# Autodesk Inventor assembly: AK80
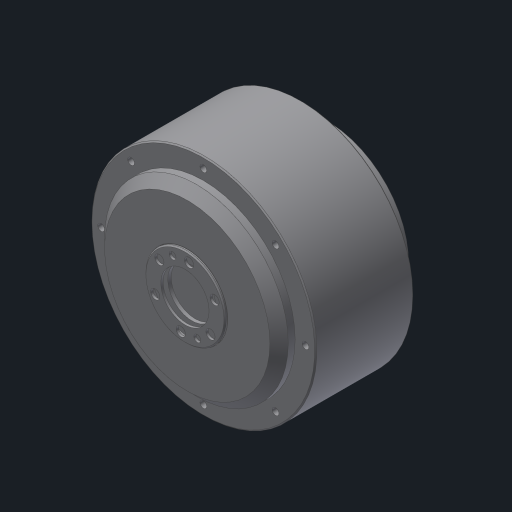
[picture p0: Inventor's stored thumbnail of the model, 512x512]
Saved by Autodesk Inventor 2023 (Build 270158000, 158)
## iProperties
Created: 2023-03-31
Part Number: AK80
Document SubType Name: Assembly
Designer: valer
Author: valer
## Documents named in this file (3)
- C:\Users\valer\Desktop\str1ker\parts\external\AK80.iam
- C:\Users\valer\Desktop\str1ker\parts\external\AK80Body.ipt
- C:\Users\valer\Desktop\str1ker\parts\external\AK80Head.ipt
## Components (2 placed, 2 different names)
1. AK80Body:1 — Mate:4, Flush:2, Flush:3, Mate:5
2. AK80Head:1 — Mate:2, Mate:5
## Relationships (5: Mate 3, Flush 2)
- Mate:2: AK80Head:1
- Mate:4: AK80Body:1
- Flush:2: AK80Body:1
- Flush:3: AK80Body:1
- Mate:5: AK80Body:1 ↔ AK80Head:1
